(part 1 of 2)
# Autodesk Inventor assembly: CNC-FullAssembly
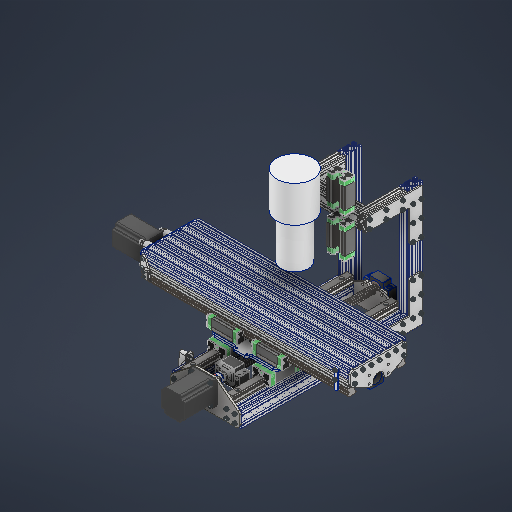
[picture p0: Inventor's stored thumbnail of the model, 512x512]
Saved by Autodesk Inventor 2026.2 (Build 302298000, 298)
## iProperties
Created: 2026-06-14
Part Number: CNC-FullAssembly
Document SubType Name: Assembly
Designer: Kenji
Mass: 17887.4 g
Surface Area: 25590.9 cm^2
Volume: 4676.24 cm^3
Density: 3.82518 g/cm^3
Author: Kenji
## Documents named in this file (45)
- C:\Users\Kenji\Documents\GitHub\DiyCNC-\CNC-FullAssembly.iam
- C:\Users\Kenji\Documents\GitHub\DiyCNC-\COTS-Parts\40x40x500mm-Extrusion.ipt
- C:\Users\Kenji\Documents\GitHub\DiyCNC-\COTS-Parts\SFU1605-BallScrewNut.iam
- C:\Users\Kenji\Documents\GitHub\DiyCNC-\COTS-Parts\DSG16H-BallScrewFixtureBlock.ipt
- C:\Users\Kenji\Documents\GitHub\DiyCNC-\COTS-Parts\SFU1605-BallScrew500mm.ipt
- C:\Users\Kenji\Documents\GitHub\DiyCNC-\COTS-Parts\BK12-BallScrewStabilizer.iam
- C:\Users\Kenji\Documents\GitHub\DiyCNC-\COTS-Parts\HGR20R-LinearRail500mm.ipt
- C:\Users\Kenji\Documents\GitHub\DiyCNC-\COTS-Parts\HGH20-LinearRailCarriage.iam
- C:\Users\Kenji\Documents\GitHub\DiyCNC-\COTS-Parts\91274A131_M5x20mm.ipt
- C:\Users\Kenji\Documents\GitHub\DiyCNC-\COTS-Parts\91290A231-M5x15mm.ipt
- C:\Users\Kenji\Documents\GitHub\DiyCNC-\COTS-Parts\Nema23-StepperMotor.ipt
- C:\Users\Kenji\Documents\GitHub\DiyCNC-\COTS-Parts\MH2025-6.35x10mmCoupler.iam
- C:\Users\Kenji\Documents\GitHub\DiyCNC-\COTS-Parts\BF12-BallScrewStabilizer2.ipt
- C:\Users\Kenji\Documents\GitHub\DiyCNC-\CNC-000-StructureGusset1.ipt
- C:\Users\Kenji\Documents\GitHub\DiyCNC-\COTS-Parts\20x40x500mm-Extrusion.ipt
- C:\Users\Kenji\Documents\GitHub\DiyCNC-\CNC-001-StructureGusset2.ipt
- C:\Users\Kenji\Documents\GitHub\DiyCNC-\CNC-002-ShimStructureGusset2.ipt
- C:\Users\Kenji\Documents\GitHub\DiyCNC-\COTS-Parts\90576A104-M5-NylockNut.ipt
- C:\Users\Kenji\Documents\GitHub\DiyCNC-\COTS-Parts\91292A195-M5x45mm.ipt
- C:\Users\Kenji\Documents\GitHub\DiyCNC-\CNC-003-StructureGusset3.ipt
- C:\Users\Kenji\Documents\GitHub\DiyCNC-\CNC-004-Nema23Shim.ipt
- C:\Users\Kenji\Documents\GitHub\DiyCNC-\COTS-Parts\91274A125-M5x8mm.ipt
- C:\Users\Kenji\Documents\GitHub\DiyCNC-\CNC-005-XAxisMount1.ipt
- C:\Users\Kenji\Documents\GitHub\DiyCNC-\COTS-Parts\91263A832-M5x10mm-Countersink.ipt
- C:\Users\Kenji\Documents\GitHub\DiyCNC-\CNC-006-XAxisMount2.ipt
- C:\Users\Kenji\Documents\GitHub\DiyCNC-\COTS-Parts\92095A495-M8-18mm-ButtonHead.ipt
- C:\Users\Kenji\Documents\GitHub\DiyCNC-\COTS-Parts\94645A210-M8-NylockNut.ipt
- C:\Users\Kenji\Documents\GitHub\DiyCNC-\COTS-Parts\20x40x500mm-Extrusion2.ipt
- C:\Users\Kenji\Documents\GitHub\DiyCNC-\COTS-Parts\20x20x500mm_Extrusion.ipt
- C:\Users\Kenji\Documents\GitHub\DiyCNC-\CNC-007-XAxisBallScrewMount.ipt
- C:\Users\Kenji\Documents\GitHub\DiyCNC-\CNC-008-XAxisNema23Mount.ipt
- C:\Users\Kenji\Documents\GitHub\DiyCNC-\CNC-009-XAxisNema23Spacer.ipt
- C:\Users\Kenji\Documents\GitHub\DiyCNC-\COTS-Parts\91290A198-M5-50mm.ipt
- C:\Users\Kenji\Documents\GitHub\DiyCNC-\COTS-Parts\3103-0001-0002-GobildaLimitSwitch.ipt
- C:\Users\Kenji\Documents\GitHub\DiyCNC-\CNC-010-XAxisLimitSwitchMount.ipt
- C:\Users\Kenji\Documents\GitHub\DiyCNC-\COTS-Parts\97763A820-M5x10mm-ButtonHead.ipt
- C:\Users\Kenji\Documents\GitHub\DiyCNC-\CNC-011-XAxisHardStop.ipt
- C:\Users\Kenji\Documents\GitHub\DiyCNC-\COTS-Parts\HGR20R-LinearRail300mm.ipt
- C:\Users\Kenji\Documents\GitHub\DiyCNC-\COTS-Parts\SFU1605-BallScrew400mm.ipt
- C:\Users\Kenji\Documents\GitHub\DiyCNC-\COTS-Parts\RouterSpindle-65mm.ipt
- C:\Users\Kenji\Documents\GitHub\DiyCNC-\COTS-Parts\90128A046-#2-.375in.ipt
- C:\Users\Kenji\Documents\GitHub\DiyCNC-\COTS-Parts\90480A003-#2-HexNut.ipt
- C:\Users\Kenji\Documents\GitHub\DiyCNC-\CNC-012-YAxisLimitSwitchMount.ipt
- C:\Users\Kenji\Documents\GitHub\DiyCNC-\COTS-Parts\20x40x100mm-Extrusion.ipt
- C:\Users\Kenji\Documents\GitHub\DiyCNC-\COTS-Parts\20x40x128mm-Extrusion.ipt
## Components (278 placed, 44 different names)
1. 40x40x500mm-Extrusion:1 — Mate:1, Mate:2, Flush:1, Flush:2, Flush:3, Angle:1, Angle:3, Angle:4, Flush:20, Flush:21, Mate:48, Mate:49, Flush:35, Mate:264, Mate:286, Flush:146, Mate:293, Tangent:7
2. 40x40x500mm-Extrusion:2 — Flush:2, Flush:3, Angle:2, Mate:39, Mate:40, Mate:41, Flush:22, Flush:23, Flush:38, Mate:290, Flush:147, Mate:294, Mate:299, Angle:12, Mate:315, Angle:13, Flush:153
3. SFU1605-BallScrewNut:1 [sub-assembly] — Mate:3, Mate:4, Mate:5, Mate:21, Mate:22, Mate:23, Mate:24, Mate:25, Mate:26, Mate:27
4. DSG16H-BallScrewFixtureBlock:1 — Mate:3, Mate:4, Mate:5, Angle:1, Flush:14, Mate:20, Angle:6, Mate:98, Mate:99
5. BK12-BallScrewStabilizer:1 [sub-assembly] — Angle:2, Mate:295, Mate:296
6. HGH20-LinearRailCarriage:1 [sub-assembly] — Flush:10, Flush:11, Mate:18, Flush:14, Mate:100, Mate:284, Mate:303, Mate:304
7. HGH20-LinearRailCarriage:2 [sub-assembly] — Flush:12, Flush:13, Mate:283, Mate:329
8. HGH20-LinearRailCarriage:3 [sub-assembly] — Flush:10, Flush:12, Mate:20, Mate:281, Mate:282, Flush:150
9. HGH20-LinearRailCarriage:4 [sub-assembly] — Flush:11, Mate:18, Flush:13, Mate:285
10. 91274A131_M5x20mm:1 — Mate:21, Mate:22, Flush:17, Flush:18
11. 91274A131_M5x20mm:2 — Mate:26, Flush:15, Flush:16
12. 91274A131_M5x20mm:3 — Mate:27, Flush:15
13. 91274A131_M5x20mm:4 — Mate:25, Flush:16, Flush:17
14. 91274A131_M5x20mm:5 — Mate:23, Flush:18, Flush:19
15. 91274A131_M5x20mm:6 — Mate:24, Flush:19
16. Nema23-StepperMotor:1 — Mate:32, Angle:3, Mate:33, Mate:59, Mate:60, Mate:61, Mate:62, Mate:63, Mate:301
17. MH2025-6.35x10mmCoupler:1 [sub-assembly] — Mate:32, Mate:33, Mate:297
18. BF12-BallScrewStabilizer2:1 — Angle:4, Mate:56, Mate:57, Mate:58, Mate:269, Mate:298
19. CNC-000-StructureGusset1:1 — Mate:39, Mate:40, Mate:41, Mate:42, Mate:43, Mate:44, Mate:45, Mate:65, Mate:77, Mate:79, Mate:265, Mate:287, Mate:291, Mate:302
20. 20x40x500mm-Extrusion:1 — Flush:20, Flush:21, Mate:71, Mate:72, Mate:73, Mate:74, Mate:75, Flush:36, Mate:293, Tangent:8, Flush:156, Flush:157, Mate:331, Flush:159, Mate:337, Mate:338, Mate:339
21. 20x40x500mm-Extrusion:2 — Flush:22, Flush:23, Mate:69, Mate:70, Mate:76, Flush:37, Mate:294, Mate:329, Mate:330, Flush:154, Flush:155, Mate:340, Mate:341
22. CNC-001-StructureGusset2:1 — Mate:48, Mate:49, Mate:51, Mate:52, Mate:53, Mate:54, Mate:55, Mate:269, Mate:299, Mate:300
23. 91290A231-M5x15mm:27 — Mate:51, Mate:52, Flush:25, Flush:26
24. 91290A231-M5x15mm:28 — Mate:54, Flush:24, Flush:25
25. 91290A231-M5x15mm:29 — Mate:55, Flush:24
26. 91290A231-M5x15mm:30 — Mate:53, Flush:26
27. CNC-002-ShimStructureGusset2:1 — Mate:56, Mate:57, Mate:58, Mate:300
28. 91274A131_M5x20mm:7 — Mate:60, Flush:29, Mate:67
29. 91274A131_M5x20mm:8 — Mate:62, Mate:63, Flush:27, Mate:68
30. 91274A131_M5x20mm:9 — Mate:59, Flush:28, Flush:29, Mate:64
31. 91274A131_M5x20mm:10 — Mate:61, Flush:27, Flush:28, Mate:66
32. 90576A104-M5-NylockNut:1 — Mate:64, Mate:65, Flush:32
33. 90576A104-M5-NylockNut:2 — Mate:66, Flush:30, Mate:78, Mate:265
34. 90576A104-M5-NylockNut:3 — Mate:68, Flush:30, Flush:31
35. 90576A104-M5-NylockNut:4 — Mate:67, Flush:31, Flush:32
36. 91292A195-M5x45mm:1 — Mate:69, Flush:33, Flush:34
37. 91292A195-M5x45mm:2 — Mate:70, Flush:34
38. 91292A195-M5x45mm:3 — Mate:72, Mate:73
39. 91292A195-M5x45mm:4 — Mate:71, Mate:74, Flush:33
40. CNC-003-StructureGusset3:1 — Mate:75, Flush:35, Flush:36, Mate:80, Mate:81, Mate:82, Mate:83
41. CNC-003-StructureGusset3:2 — Mate:76, Flush:37, Flush:38, Mate:84, Mate:85, Mate:86, Mate:87
42. CNC-004-Nema23Shim:1 — Mate:77, Mate:78, Mate:79, Mate:301
43. HGH20-LinearRailCarriage:5 [sub-assembly] — Mate:91, Mate:92, Mate:131, Mate:132, Mate:133, Flush:142
44. HGH20-LinearRailCarriage:6 [sub-assembly] — Mate:128, Mate:129, Mate:130
45. HGH20-LinearRailCarriage:7 [sub-assembly] — Mate:125, Mate:126, Mate:127
46. HGH20-LinearRailCarriage:8 [sub-assembly] — Mate:134, Mate:135, Mate:136, Mate:137, Mate:138
47. HGR20R-LinearRail500mm:3 — Flush:50, Mate:137, Mate:138, Mate:202, Mate:226, Mate:314
48. HGR20R-LinearRail500mm:4 — Mate:91, Mate:92, Flush:50, Flush:106, Flush:107, Mate:199, Flush:119, Angle:10, Mate:224, Mate:225, Flush:142, Mate:313
49. DSG16H-BallScrewFixtureBlock:2 — Angle:6, Mate:94, Mate:95, Mate:96, Mate:97, Mate:121, Mate:122, Mate:123
50. SFU1605-BallScrewNut:2 [sub-assembly] — Mate:94, Mate:95, Mate:96, Mate:139, Mate:140, Mate:141, Mate:142, Mate:143, Mate:144, Mate:145
51. SFU1605-BallScrew500mm:2 — Mate:97, Mate:203, Mate:204, Mate:205, Mate:207, Mate:209, Mate:256
52. CNC-005-XAxisMount1:1 — Mate:98, Mate:99, Mate:100, Mate:101, Flush:53, Mate:102, Mate:103, Mate:104, Mate:105, Mate:106, Mate:107, Mate:108, Flush:57, Flush:58, Flush:59, Flush:60, Mate:109, Mate:110, Mate:111, Mate:112, Flush:61, Flush:63, Mate:113, Mate:114, Mate:115, Mate:116, Flush:65, Flush:66, Flush:67, Flush:68, Mate:117, Mate:118, Mate:119, Mate:120, Flush:69, Flush:70, Flush:71, Flush:72, Mate:124, Angle:7, Mate:166, Mate:177, Mate:179, Mate:181, Mate:183, Mate:186, Mate:187, Mate:190, Mate:191, Mate:282, Mate:283, Mate:285
53. 91263A832-M5x10mm-Countersink:1 — Mate:101, Flush:53, Flush:56
54. 91263A832-M5x10mm-Countersink:2 — Mate:104, Flush:55, Mate:281
55. 91263A832-M5x10mm-Countersink:3 — Mate:102, Flush:54, Flush:55, Flush:56
56. 91263A832-M5x10mm-Countersink:4 — Mate:103, Flush:54
57. 91263A832-M5x10mm-Countersink:5 — Mate:105, Flush:59
58. 91263A832-M5x10mm-Countersink:6 — Mate:106, Flush:58, Mate:284
59. 91263A832-M5x10mm-Countersink:7 — Mate:108, Flush:57
60. 91263A832-M5x10mm-Countersink:8 — Mate:107, Flush:60
61. 91263A832-M5x10mm-Countersink:9 — Mate:112, Flush:62
62. 91263A832-M5x10mm-Countersink:10 — Mate:111, Flush:61, Flush:62
63. 91263A832-M5x10mm-Countersink:11 — Mate:109, Flush:63, Flush:64
64. 91263A832-M5x10mm-Countersink:12 — Mate:110, Flush:64
65. 91263A832-M5x10mm-Countersink:13 — Mate:113, Flush:65
66. 91263A832-M5x10mm-Countersink:14 — Mate:116, Flush:67
67. 91263A832-M5x10mm-Countersink:15 — Mate:115, Flush:66
68. 91263A832-M5x10mm-Countersink:16 — Mate:114, Flush:68
69. 91263A832-M5x10mm-Countersink:17 — Mate:118, Flush:71
70. 91263A832-M5x10mm-Countersink:18 — Mate:119, Flush:69
71. 91263A832-M5x10mm-Countersink:19 — Mate:117, Flush:72
72. 91263A832-M5x10mm-Countersink:20 — Mate:120, Flush:70
73. CNC-006-XAxisMount2:1 — Mate:121, Mate:122, Mate:123, Mate:124, Angle:7, Mate:125, Mate:126, Mate:127, Mate:128, Mate:129, Mate:130, Mate:131, Mate:132, Mate:133, Mate:134, Mate:135, Mate:136, Mate:146, Mate:147, Mate:148, Mate:149, Flush:78, Flush:79, Flush:81, Mate:150, Mate:151, Mate:152, Mate:153, Flush:82, Flush:83, Flush:84, Flush:85, Mate:154, Mate:155, Mate:156, Mate:157, Flush:86, Flush:87, Mate:158, Mate:159, Mate:160, Mate:161, Flush:90, Flush:91, Flush:92, Flush:93, Mate:162, Mate:163, Mate:164, Mate:165, Flush:94, Flush:95, Flush:96, Flush:97, Mate:166, Mate:167, Mate:168, Mate:169, Mate:170, Mate:171, Mate:172, Mate:173, Mate:174, Mate:175
74. 91274A131_M5x20mm:11 — Mate:139, Mate:140, Flush:74, Flush:75
75. 91274A131_M5x20mm:12 — Mate:145, Flush:76, Flush:77
76. 91274A131_M5x20mm:13 — Mate:144, Flush:77
77. 91274A131_M5x20mm:14 — Mate:141, Flush:73, Flush:74
78. 91274A131_M5x20mm:15 — Mate:143, Flush:75
79. 91274A131_M5x20mm:16 — Mate:142, Flush:73, Flush:76
80. 91263A832-M5x10mm-Countersink:21 — Mate:149, Flush:78
81. 91263A832-M5x10mm-Countersink:22 — Mate:146, Flush:80
82. 91263A832-M5x10mm-Countersink:23 — Mate:147, Flush:79, Flush:80
83. 91263A832-M5x10mm-Countersink:24 — Mate:148, Flush:81
84. 91263A832-M5x10mm-Countersink:25 — Mate:150, Flush:85
85. 91263A832-M5x10mm-Countersink:26 — Mate:153, Flush:83
86. 91263A832-M5x10mm-Countersink:27 — Mate:151, Flush:82
87. 91263A832-M5x10mm-Countersink:28 — Mate:152, Flush:84
88. 91263A832-M5x10mm-Countersink:29 — Mate:156, Flush:87, Flush:88
89. 91263A832-M5x10mm-Countersink:30 — Mate:155, Flush:89
90. 91263A832-M5x10mm-Countersink:31 — Mate:154, Flush:88, Flush:89
91. 91263A832-M5x10mm-Countersink:32 — Mate:157, Flush:86
92. 91263A832-M5x10mm-Countersink:33 — Mate:159, Flush:93
93. 91263A832-M5x10mm-Countersink:34 — Mate:160, Flush:91
94. 91263A832-M5x10mm-Countersink:35 — Mate:158, Flush:92
95. 91263A832-M5x10mm-Countersink:36 — Mate:161, Flush:90
96. 91263A832-M5x10mm-Countersink:37 — Mate:164, Flush:95
97. 91263A832-M5x10mm-Countersink:38 — Mate:162, Flush:96
98. 91263A832-M5x10mm-Countersink:39 — Mate:163, Flush:97
99. 91263A832-M5x10mm-Countersink:40 — Mate:165, Flush:94
100. 92095A495-M8-18mm-ButtonHead:1 — Mate:167, Flush:98, Flush:99, Flush:102, Mate:176
101. 92095A495-M8-18mm-ButtonHead:2 — Mate:168, Flush:99, Flush:104, Mate:178
102. 92095A495-M8-18mm-ButtonHead:3 — Mate:169, Mate:170, Flush:98, Flush:100, Mate:180
103. 92095A495-M8-18mm-ButtonHead:8 — Mate:171, Flush:100, Mate:182
104. 92095A495-M8-18mm-ButtonHead:9 — Mate:174, Flush:103, Flush:104, Mate:188
105. 92095A495-M8-18mm-ButtonHead:10 — Mate:175, Flush:103, Mate:189
106. 92095A495-M8-18mm-ButtonHead:11 — Mate:172, Flush:101, Flush:102, Mate:184
107. 92095A495-M8-18mm-ButtonHead:12 — Mate:173, Flush:101, Mate:185
108. 94645A210-M8-NylockNut:1 — Mate:176, Mate:177
109. 94645A210-M8-NylockNut:2 — Mate:178, Mate:179
110. 94645A210-M8-NylockNut:3 — Mate:180, Mate:181
111. 94645A210-M8-NylockNut:4 — Mate:182, Mate:183
112. 94645A210-M8-NylockNut:5 — Mate:184, Mate:187
113. 94645A210-M8-NylockNut:6 — Mate:185, Mate:186
114. 94645A210-M8-NylockNut:7 — Mate:188, Mate:191
115. 94645A210-M8-NylockNut:8 — Mate:189, Mate:190
116. 20x40x500mm-Extrusion2:1 — Flush:106, Flush:107, Flush:108, Mate:193, Flush:109, Flush:116, Flush:117, Mate:200, Mate:211, Mate:212, Mate:213, Angle:11, Tangent:2, Flush:143, Tangent:4, Mate:270
117. 20x40x500mm-Extrusion2:2 — Flush:108, Mate:193, Flush:109, Flush:110, Flush:111, Mate:194, Angle:8, Angle:9
118. 20x40x500mm-Extrusion2:3 — Flush:110, Flush:111, Mate:194, Mate:201, Flush:118, Mate:228, Mate:229
119. 20x20x500mm_Extrusion:3 — Flush:116, Mate:199, Flush:117, Mate:200, Tangent:3, Tangent:5, Flush:144, Mate:312
120. 20x40x500mm-Extrusion2:4 — Mate:201, Flush:118, Mate:202, Mate:227, Mate:276
121. BF12-BallScrewStabilizer2:2 — Mate:203, Mate:204, Flush:119, Angle:8
122. Nema23-StepperMotor:2 — Mate:205, Angle:9, Mate:206, Mate:208, Mate:243, Mate:244, Mate:245, Mate:246, Mate:247
123. MH2025-6.35x10mmCoupler:2 [sub-assembly] — Mate:206, Mate:207, Mate:208, Mate:240
124. BK12-BallScrewStabilizer:2 [sub-assembly] — Mate:209, Angle:10, Mate:256
125. CNC-007-XAxisBallScrewMount:1 — Mate:211, Mate:212, Mate:213, Mate:214, Mate:215, Mate:216, Mate:217, Mate:218, Mate:219, Mate:220, Mate:221, Mate:222, Mate:223
126. 91290A231-M5x15mm:31 — Mate:219, Flush:123, Flush:124
127. 91290A231-M5x15mm:32 — Mate:218, Flush:122, Flush:123, Flush:125, Flush:127
128. 91290A231-M5x15mm:33 — Mate:215, Flush:120, Flush:121
129. 91290A231-M5x15mm:34 — Mate:216, Flush:120
130. 91290A231-M5x15mm:35 — Mate:220, Flush:124
131. 91290A231-M5x15mm:36 — Mate:214, Mate:221, Flush:125, Flush:126
132. 91290A231-M5x15mm:37 — Mate:217, Flush:121, Flush:122
133. 91290A231-M5x15mm:38 — Mate:222, Flush:126
134. 91290A231-M5x15mm:39 — Mate:223, Flush:127
135. CNC-008-XAxisNema23Mount:1 — Mate:227, Mate:228, Mate:229, Mate:230, Mate:231, Mate:232, Mate:233, Mate:234, Mate:235, Mate:236, Mate:237, Mate:238, Mate:239, Mate:241, Mate:242, Mate:252, Mate:253, Mate:254, Mate:255
136. 91290A231-M5x15mm:58 — Mate:233, Flush:133, Flush:134
137. 91290A231-M5x15mm:59 — Mate:231, Flush:134, Flush:135
138. 91290A231-M5x15mm:60 — Mate:232, Flush:136
139. 91290A231-M5x15mm:61 — Mate:234, Flush:132, Flush:133
140. 91290A231-M5x15mm:62 — Mate:235, Flush:131, Flush:132
141. 91290A231-M5x15mm:63 — Mate:238, Mate:239, Flush:129
142. 91290A231-M5x15mm:64 — Mate:230, Flush:135, Flush:136
143. 91290A231-M5x15mm:65 — Mate:237, Flush:129, Flush:130
144. 91290A231-M5x15mm:66 — Mate:236, Flush:130, Flush:131
145. CNC-009-XAxisNema23Spacer:1 — Mate:240, Mate:241, Mate:242
146. 91290A198-M5-50mm:1 — Mate:244, Flush:138, Mate:248
147. 91290A198-M5-50mm:2 — Mate:243, Flush:138, Flush:139, Mate:250
148. 91290A198-M5-50mm:3 — Mate:245, Flush:137, Flush:139, Mate:251
149. 91290A198-M5-50mm:4 — Mate:246, Mate:247, Flush:137, Mate:249
150. 90576A104-M5-NylockNut:5 — Mate:251, Mate:252
151. 90576A104-M5-NylockNut:6 — Mate:248, Mate:254
152. 90576A104-M5-NylockNut:7 — Mate:250, Mate:255
153. 90576A104-M5-NylockNut:8 — Mate:249, Mate:253
154. 3103-0001-0002-GobildaLimitSwitch:1 — Angle:11, Mate:258, Mate:259, Mate:305, Mate:306, Mate:310
155. CNC-010-XAxisLimitSwitchMount:1 — Tangent:2, Mate:258, Mate:259, Mate:260, Mate:261, Mate:262, Mate:263, Tangent:3, Flush:143, Mate:307, Mate:308, Mate:312
156. 97763A820-M5x10mm-ButtonHead:1 — Mate:262, Mate:263
157. 97763A820-M5x10mm-ButtonHead:2 — Mate:260, Mate:261
158. CNC-011-XAxisHardStop:1 — Tangent:4, Tangent:5, Mate:270, Flush:144, Mate:271, Mate:272, Mate:273, Mate:274
159. 91274A125-M5x8mm:25 — Mate:271, Mate:272, Flush:145
160. 91274A125-M5x8mm:26 — Mate:273, Flush:145, Mate:275
161. CNC-011-XAxisHardStop:2 — Mate:274, Mate:275, Mate:276, Mate:277, Mate:278, Mate:279, Mate:280
162. 91274A125-M5x8mm:27 — Mate:277, Mate:280
163. 91274A125-M5x8mm:28 — Mate:278, Mate:279
164. HGR20R-LinearRail300mm:1 — Mate:290, Mate:291, Flush:147, Mate:292
165. HGR20R-LinearRail300mm:2 — Mate:286, Flush:146, Mate:287, Mate:288, Mate:289, Mate:303, Mate:304
166. SFU1605-BallScrew400mm:1 — Mate:295, Mate:296, Mate:297, Mate:298
167. RouterSpindle-65mm:1 — Tangent:7, Tangent:8
168. 90128A046-#2-.375in:1 — Mate:305, Mate:308, Mate:311
169. 90128A046-#2-.375in:2 — Mate:306, Mate:307, Mate:309
170. 90480A003-#2-HexNut:1 — Mate:309, Mate:310, Flush:149
171. 90480A003-#2-HexNut:2 — Mate:311, Flush:149
172. 3103-0001-0002-GobildaLimitSwitch:2 — Angle:12, Flush:150, Mate:315, Mate:316, Mate:318, Mate:321, Mate:323, Mate:324, Mate:325
173. CNC-012-YAxisLimitSwitchMount:1 — Mate:316, Mate:318, Angle:13, Mate:319, Angle:14, Mate:320, Angle:15, Mate:322, Mate:326, Mate:327, Mate:328, Flush:153
174. 90480A003-#2-HexNut:3 — Mate:319, Angle:14, Mate:320
175. 90480A003-#2-HexNut:4 — Mate:321, Angle:15, Mate:322
176. 90128A046-#2-.375in:3 — Mate:323, Flush:151
177. 90128A046-#2-.375in:4 — Mate:324, Mate:325, Flush:151
178. 97763A820-M5x10mm-ButtonHead:3 — Mate:326, Flush:152
179. 97763A820-M5x10mm-ButtonHead:4 — Mate:327, Mate:328, Flush:152
180. 20x40x100mm-Extrusion:3 — Mate:330, Flush:154, Flush:155, Mate:335, Mate:336, Flush:160, Flush:161
181. 20x40x100mm-Extrusion:4 — Flush:156, Flush:157, Mate:331, Mate:332, Flush:158
182. CNC-003-StructureGusset3:3 — Mate:332, Flush:158, Flush:159, Mate:333, Mate:334, Mate:342, Mate:343, Mate:344
183. CNC-003-StructureGusset3:4 — Mate:333, Mate:334, Mate:335, Mate:345, Mate:346, Mate:347, Mate:348
184. 20x40x128mm-Extrusion:1 — Mate:336, Flush:160, Flush:161, Mate:349, Angle:16, Flush:168, Mate:350
185. 91292A195-M5x45mm:5 — Mate:337, Mate:338, Flush:164
186. 91292A195-M5x45mm:6 — Mate:341, Flush:162
187. 91292A195-M5x45mm:7 — Mate:339, Flush:163, Flush:164
188. 91292A195-M5x45mm:8 — Mate:340, Flush:162, Flush:163
189. HGH20-LinearRailCarriage:9 [sub-assembly] — Mate:349, Angle:16, Flush:166, Flush:167, Mate:351
190. HGH20-LinearRailCarriage:10 [sub-assembly] — Flush:166, Flush:167, Flush:168, Mate:350, Mate:351
191. 91290A231-M5x15mm:20 — Mate:44, Mate:45
192. 91290A231-M5x15mm:21
193. 91290A231-M5x15mm:22 — Mate:264
194. 91290A231-M5x15mm:23 — Mate:302
195. 91290A231-M5x15mm:19 — Mate:42, Mate:43
196. 91290A231-M5x15mm:24
197. 91290A231-M5x15mm:25
198. 91290A231-M5x15mm:26
199. 91274A125-M5x8mm:1 — Mate:80, Mate:81
200. 91274A125-M5x8mm:2
201. 91274A125-M5x8mm:3
202. 91274A125-M5x8mm:4
203. 91274A125-M5x8mm:5
204. 91274A125-M5x8mm:6
205. 91274A125-M5x8mm:7 — Mate:82, Mate:83
206. 91274A125-M5x8mm:8
207. 91274A125-M5x8mm:9
208. 91274A125-M5x8mm:10
209. 91274A125-M5x8mm:11
210. 91274A125-M5x8mm:12
211. 91274A125-M5x8mm:13 — Mate:84, Mate:85
212. 91274A125-M5x8mm:14
213. 91274A125-M5x8mm:15
214. 91274A125-M5x8mm:16
215. 91274A125-M5x8mm:17
216. 91274A125-M5x8mm:18
217. 91274A125-M5x8mm:19 — Mate:86, Mate:87
218. 91274A125-M5x8mm:20
219. 91274A125-M5x8mm:21
220. 91274A125-M5x8mm:22
221. 91274A125-M5x8mm:23
222. 91274A125-M5x8mm:24
223. 91290A231-M5x15mm:41 — Mate:226, Flush:128
224. 91290A231-M5x15mm:40 — Mate:224, Mate:225, Flush:128
225. 91290A231-M5x15mm:67
226. 91290A231-M5x15mm:68
227. 91290A231-M5x15mm:69
228. 91290A231-M5x15mm:70
229. 91290A231-M5x15mm:71
230. 91290A231-M5x15mm:72
231. 91290A231-M5x15mm:73
232. 91290A231-M5x15mm:74
233. 91290A231-M5x15mm:75
234. 91290A231-M5x15mm:76
235. 91290A231-M5x15mm:77
236. 91290A231-M5x15mm:78
237. 91290A231-M5x15mm:79
238. 91290A231-M5x15mm:80
239. 91290A231-M5x15mm:81 — Mate:314
240. 91290A231-M5x15mm:82 — Mate:313
241. 91290A231-M5x15mm:83 — Mate:292, Flush:148
242. 91290A231-M5x15mm:1 — Mate:288, Mate:289, Flush:148
243. 91290A231-M5x15mm:84
244. 91290A231-M5x15mm:85
245. 91290A231-M5x15mm:86
246. 91290A231-M5x15mm:87
247. 91290A231-M5x15mm:88
248. 91290A231-M5x15mm:89
249. 91290A231-M5x15mm:90
250. 91290A231-M5x15mm:91
251. 91290A231-M5x15mm:92
252. 91290A231-M5x15mm:93
253. 91290A231-M5x15mm:94
254. 91290A231-M5x15mm:95
255. 91274A125-M5x8mm:29 — Mate:342, Mate:343, Flush:165
256. 91274A125-M5x8mm:33
257. 91274A125-M5x8mm:34
258. 91274A125-M5x8mm:35
259. 91274A125-M5x8mm:36
260. 91274A125-M5x8mm:37
261. 91274A125-M5x8mm:30 — Mate:344, Flush:165
262. 91274A125-M5x8mm:38
263. 91274A125-M5x8mm:39
264. 91274A125-M5x8mm:40
265. 91274A125-M5x8mm:41
266. 91274A125-M5x8mm:42
267. 91274A125-M5x8mm:31 — Mate:345, Mate:346
268. 91274A125-M5x8mm:43
269. 91274A125-M5x8mm:44
270. 91274A125-M5x8mm:45
271. 91274A125-M5x8mm:46
272. 91274A125-M5x8mm:47
273. 91274A125-M5x8mm:32 — Mate:347, Mate:348
274. 91274A125-M5x8mm:48
275. 91274A125-M5x8mm:49
276. 91274A125-M5x8mm:50
277. 91274A125-M5x8mm:51
278. 91274A125-M5x8mm:52
## Component patterns: (4 elements, first: 91290A231-M5x15mm:20), (4 elements, first: 91290A231-M5x15mm:19), (6 elements, first: 91274A125-M5x8mm:1), (6 elements, first: 91274A125-M5x8mm:7), (6 elements, first: 91274A125-M5x8mm:13), (6 elements, first: 91274A125-M5x8mm:19), (9 elements, first: 91290A231-M5x15mm:41 + 91290A231-M5x15mm:40), (7 elements, first: 91290A231-M5x15mm:83 + 91290A231-M5x15mm:1), (6 elements, first: 91274A125-M5x8mm:29), (6 elements, first: 91274A125-M5x8mm:30), (6 elements, first: 91274A125-M5x8mm:31), (6 elements, first: 91274A125-M5x8mm:32)
## Relationships (474: Mate 311, Flush 142, Angle 15, Tangent 6)
- Mate:1 (-20 mm): 40x40x500mm-Extrusion:1
- Mate:2 (-20 mm): 40x40x500mm-Extrusion:1
- Flush:1 (-250 mm): 40x40x500mm-Extrusion:1
- Flush:2: 40x40x500mm-Extrusion:1 ↔ 40x40x500mm-Extrusion:2
- Flush:3: 40x40x500mm-Extrusion:1 ↔ 40x40x500mm-Extrusion:2
- Mate:3: SFU1605-BallScrewNut:1 ↔ DSG16H-BallScrewFixtureBlock:1
- Mate:4: SFU1605-BallScrewNut:1 ↔ DSG16H-BallScrewFixtureBlock:1
- Mate:5: SFU1605-BallScrewNut:1 ↔ DSG16H-BallScrewFixtureBlock:1
- Angle:1 (0 deg): 40x40x500mm-Extrusion:1 ↔ DSG16H-BallScrewFixtureBlock:1
- Angle:2 (0 deg): 40x40x500mm-Extrusion:2 ↔ BK12-BallScrewStabilizer:1
- Flush:10: HGH20-LinearRailCarriage:1 ↔ HGH20-LinearRailCarriage:3
- Flush:11: HGH20-LinearRailCarriage:1 ↔ HGH20-LinearRailCarriage:4
- Mate:18 (40 mm): HGH20-LinearRailCarriage:1 ↔ HGH20-LinearRailCarriage:4
- Flush:12: HGH20-LinearRailCarriage:2 ↔ HGH20-LinearRailCarriage:3
- Flush:13: HGH20-LinearRailCarriage:2 ↔ HGH20-LinearRailCarriage:4
- Flush:14: DSG16H-BallScrewFixtureBlock:1 ↔ HGH20-LinearRailCarriage:1
- Mate:20: DSG16H-BallScrewFixtureBlock:1 ↔ HGH20-LinearRailCarriage:3
- Mate:21: SFU1605-BallScrewNut:1 ↔ 91274A131_M5x20mm:1
- Mate:22: SFU1605-BallScrewNut:1 ↔ 91274A131_M5x20mm:1
- Mate:23: SFU1605-BallScrewNut:1 ↔ 91274A131_M5x20mm:5
- Mate:24: SFU1605-BallScrewNut:1 ↔ 91274A131_M5x20mm:6
- Mate:25: SFU1605-BallScrewNut:1 ↔ 91274A131_M5x20mm:4
- Mate:26: SFU1605-BallScrewNut:1 ↔ 91274A131_M5x20mm:2
- Mate:27: SFU1605-BallScrewNut:1 ↔ 91274A131_M5x20mm:3
- Flush:15: 91274A131_M5x20mm:2 ↔ 91274A131_M5x20mm:3
- Flush:16: 91274A131_M5x20mm:2 ↔ 91274A131_M5x20mm:4
- Flush:17: 91274A131_M5x20mm:1 ↔ 91274A131_M5x20mm:4
- Flush:18: 91274A131_M5x20mm:1 ↔ 91274A131_M5x20mm:5
- Flush:19: 91274A131_M5x20mm:5 ↔ 91274A131_M5x20mm:6
- Mate:32: Nema23-StepperMotor:1 ↔ MH2025-6.35x10mmCoupler:1
- Angle:3 (0 deg): 40x40x500mm-Extrusion:1 ↔ Nema23-StepperMotor:1
- Mate:33 (2 mm): Nema23-StepperMotor:1 ↔ MH2025-6.35x10mmCoupler:1
- Angle:4 (0 deg): 40x40x500mm-Extrusion:1 ↔ BF12-BallScrewStabilizer2:1
- Mate:39: 40x40x500mm-Extrusion:2 ↔ CNC-000-StructureGusset1:1
- Mate:40: 40x40x500mm-Extrusion:2 ↔ CNC-000-StructureGusset1:1
- Mate:41: 40x40x500mm-Extrusion:2 ↔ CNC-000-StructureGusset1:1
- Mate:42: CNC-000-StructureGusset1:1 ↔ 91290A231-M5x15mm:19
- Mate:43: CNC-000-StructureGusset1:1 ↔ 91290A231-M5x15mm:19
- Mate:44: CNC-000-StructureGusset1:1 ↔ 91290A231-M5x15mm:20
- Mate:45: CNC-000-StructureGusset1:1 ↔ 91290A231-M5x15mm:20
- Flush:20: 40x40x500mm-Extrusion:1 ↔ 20x40x500mm-Extrusion:1
- Flush:21: 40x40x500mm-Extrusion:1 ↔ 20x40x500mm-Extrusion:1
- Flush:22: 40x40x500mm-Extrusion:2 ↔ 20x40x500mm-Extrusion:2
- Flush:23: 40x40x500mm-Extrusion:2 ↔ 20x40x500mm-Extrusion:2
- Mate:48: 40x40x500mm-Extrusion:1 ↔ CNC-001-StructureGusset2:1
- Mate:49: 40x40x500mm-Extrusion:1 ↔ CNC-001-StructureGusset2:1
- Mate:51: CNC-001-StructureGusset2:1 ↔ 91290A231-M5x15mm:27
- Mate:52: CNC-001-StructureGusset2:1 ↔ 91290A231-M5x15mm:27
- Mate:53: CNC-001-StructureGusset2:1 ↔ 91290A231-M5x15mm:30
- Mate:54: CNC-001-StructureGusset2:1 ↔ 91290A231-M5x15mm:28
- Mate:55: CNC-001-StructureGusset2:1 ↔ 91290A231-M5x15mm:29
- Flush:24: 91290A231-M5x15mm:28 ↔ 91290A231-M5x15mm:29
- Flush:25: 91290A231-M5x15mm:27 ↔ 91290A231-M5x15mm:28
- Flush:26: 91290A231-M5x15mm:27 ↔ 91290A231-M5x15mm:30
- Mate:56: BF12-BallScrewStabilizer2:1 ↔ CNC-002-ShimStructureGusset2:1
- Mate:57: BF12-BallScrewStabilizer2:1 ↔ CNC-002-ShimStructureGusset2:1
- Mate:58: BF12-BallScrewStabilizer2:1 ↔ CNC-002-ShimStructureGusset2:1
- Mate:59: Nema23-StepperMotor:1 ↔ 91274A131_M5x20mm:9
- Mate:60: Nema23-StepperMotor:1 ↔ 91274A131_M5x20mm:7
- Mate:61: Nema23-StepperMotor:1 ↔ 91274A131_M5x20mm:10
- Mate:62: Nema23-StepperMotor:1 ↔ 91274A131_M5x20mm:8
- Mate:63: Nema23-StepperMotor:1 ↔ 91274A131_M5x20mm:8
- Flush:27: 91274A131_M5x20mm:8 ↔ 91274A131_M5x20mm:10
- Flush:28: 91274A131_M5x20mm:9 ↔ 91274A131_M5x20mm:10
- Flush:29: 91274A131_M5x20mm:7 ↔ 91274A131_M5x20mm:9
- Mate:64: 91274A131_M5x20mm:9 ↔ 90576A104-M5-NylockNut:1
- Mate:65: CNC-000-StructureGusset1:1 ↔ 90576A104-M5-NylockNut:1
- Mate:66: 91274A131_M5x20mm:10 ↔ 90576A104-M5-NylockNut:2
- Mate:67: 91274A131_M5x20mm:7 ↔ 90576A104-M5-NylockNut:4
- Mate:68: 91274A131_M5x20mm:8 ↔ 90576A104-M5-NylockNut:3
- Flush:30: 90576A104-M5-NylockNut:2 ↔ 90576A104-M5-NylockNut:3
- Flush:31: 90576A104-M5-NylockNut:3 ↔ 90576A104-M5-NylockNut:4
- Flush:32: 90576A104-M5-NylockNut:1 ↔ 90576A104-M5-NylockNut:4
- Mate:69: 20x40x500mm-Extrusion:2 ↔ 91292A195-M5x45mm:1
- Mate:70: 20x40x500mm-Extrusion:2 ↔ 91292A195-M5x45mm:2
- Mate:71: 20x40x500mm-Extrusion:1 ↔ 91292A195-M5x45mm:4
- Mate:72: 20x40x500mm-Extrusion:1 ↔ 91292A195-M5x45mm:3
- Mate:73: 20x40x500mm-Extrusion:1 ↔ 91292A195-M5x45mm:3
- Mate:74: 20x40x500mm-Extrusion:1 ↔ 91292A195-M5x45mm:4
- Flush:33: 91292A195-M5x45mm:1 ↔ 91292A195-M5x45mm:4
- Flush:34: 91292A195-M5x45mm:1 ↔ 91292A195-M5x45mm:2
- Mate:75: 20x40x500mm-Extrusion:1 ↔ CNC-003-StructureGusset3:1
- Flush:35 (4.225 mm): 40x40x500mm-Extrusion:1 ↔ CNC-003-StructureGusset3:1
- Flush:36 (-4.225 mm): 20x40x500mm-Extrusion:1 ↔ CNC-003-StructureGusset3:1
- Mate:76: 20x40x500mm-Extrusion:2 ↔ CNC-003-StructureGusset3:2
- Flush:37 (-4.225 mm): 20x40x500mm-Extrusion:2 ↔ CNC-003-StructureGusset3:2
- Flush:38 (4.225 mm): 40x40x500mm-Extrusion:2 ↔ CNC-003-StructureGusset3:2
- Mate:77: CNC-000-StructureGusset1:1 ↔ CNC-004-Nema23Shim:1
- Mate:78: 90576A104-M5-NylockNut:2 ↔ CNC-004-Nema23Shim:1
- Mate:79: CNC-000-StructureGusset1:1 ↔ CNC-004-Nema23Shim:1
- Mate:80: CNC-003-StructureGusset3:1 ↔ 91274A125-M5x8mm:1
- Mate:81: CNC-003-StructureGusset3:1 ↔ 91274A125-M5x8mm:1
- Mate:82: CNC-003-StructureGusset3:1 ↔ 91274A125-M5x8mm:7
- Mate:83: CNC-003-StructureGusset3:1 ↔ 91274A125-M5x8mm:7
- Mate:84: CNC-003-StructureGusset3:2 ↔ 91274A125-M5x8mm:13
- Mate:85: CNC-003-StructureGusset3:2 ↔ 91274A125-M5x8mm:13
- Mate:86: CNC-003-StructureGusset3:2 ↔ 91274A125-M5x8mm:19
- Mate:87: CNC-003-StructureGusset3:2 ↔ 91274A125-M5x8mm:19
- Mate:91: HGH20-LinearRailCarriage:5 ↔ HGR20R-LinearRail500mm:4
- Mate:92: HGH20-LinearRailCarriage:5 ↔ HGR20R-LinearRail500mm:4
- Flush:50: HGR20R-LinearRail500mm:3 ↔ HGR20R-LinearRail500mm:4
- Angle:6 (180 deg): DSG16H-BallScrewFixtureBlock:1 ↔ DSG16H-BallScrewFixtureBlock:2
- Mate:94: DSG16H-BallScrewFixtureBlock:2 ↔ SFU1605-BallScrewNut:2
- Mate:95: DSG16H-BallScrewFixtureBlock:2 ↔ SFU1605-BallScrewNut:2
- Mate:96: DSG16H-BallScrewFixtureBlock:2 ↔ SFU1605-BallScrewNut:2
- Mate:97: DSG16H-BallScrewFixtureBlock:2 ↔ SFU1605-BallScrew500mm:2
- Mate:98: DSG16H-BallScrewFixtureBlock:1 ↔ CNC-005-XAxisMount1:1
- Mate:99: DSG16H-BallScrewFixtureBlock:1 ↔ CNC-005-XAxisMount1:1
- Mate:100: HGH20-LinearRailCarriage:1 ↔ CNC-005-XAxisMount1:1
- Mate:101: CNC-005-XAxisMount1:1 ↔ 91263A832-M5x10mm-Countersink:1
- Flush:53: CNC-005-XAxisMount1:1 ↔ 91263A832-M5x10mm-Countersink:1
- Mate:102: CNC-005-XAxisMount1:1 ↔ 91263A832-M5x10mm-Countersink:3
- Mate:103: CNC-005-XAxisMount1:1 ↔ 91263A832-M5x10mm-Countersink:4
- Mate:104: CNC-005-XAxisMount1:1 ↔ 91263A832-M5x10mm-Countersink:2
- Flush:54: 91263A832-M5x10mm-Countersink:3 ↔ 91263A832-M5x10mm-Countersink:4
- Flush:55: 91263A832-M5x10mm-Countersink:2 ↔ 91263A832-M5x10mm-Countersink:3
- Flush:56: 91263A832-M5x10mm-Countersink:1 ↔ 91263A832-M5x10mm-Countersink:3
- Mate:105: CNC-005-XAxisMount1:1 ↔ 91263A832-M5x10mm-Countersink:5
- Mate:106: CNC-005-XAxisMount1:1 ↔ 91263A832-M5x10mm-Countersink:6
- Mate:107: CNC-005-XAxisMount1:1 ↔ 91263A832-M5x10mm-Countersink:8
- Mate:108: CNC-005-XAxisMount1:1 ↔ 91263A832-M5x10mm-Countersink:7
- Flush:57: CNC-005-XAxisMount1:1 ↔ 91263A832-M5x10mm-Countersink:7
- Flush:58: CNC-005-XAxisMount1:1 ↔ 91263A832-M5x10mm-Countersink:6
- Flush:59: CNC-005-XAxisMount1:1 ↔ 91263A832-M5x10mm-Countersink:5
- Flush:60: CNC-005-XAxisMount1:1 ↔ 91263A832-M5x10mm-Countersink:8
- Mate:109: CNC-005-XAxisMount1:1 ↔ 91263A832-M5x10mm-Countersink:11
- Mate:110: CNC-005-XAxisMount1:1 ↔ 91263A832-M5x10mm-Countersink:12
- Mate:111: CNC-005-XAxisMount1:1 ↔ 91263A832-M5x10mm-Countersink:10
- Mate:112: CNC-005-XAxisMount1:1 ↔ 91263A832-M5x10mm-Countersink:9
- Flush:61: CNC-005-XAxisMount1:1 ↔ 91263A832-M5x10mm-Countersink:10
- Flush:62: 91263A832-M5x10mm-Countersink:9 ↔ 91263A832-M5x10mm-Countersink:10
- Flush:63: CNC-005-XAxisMount1:1 ↔ 91263A832-M5x10mm-Countersink:11
- Flush:64: 91263A832-M5x10mm-Countersink:11 ↔ 91263A832-M5x10mm-Countersink:12
- Mate:113: CNC-005-XAxisMount1:1 ↔ 91263A832-M5x10mm-Countersink:13
- Mate:114: CNC-005-XAxisMount1:1 ↔ 91263A832-M5x10mm-Countersink:16
- Mate:115: CNC-005-XAxisMount1:1 ↔ 91263A832-M5x10mm-Countersink:15
- Mate:116: CNC-005-XAxisMount1:1 ↔ 91263A832-M5x10mm-Countersink:14
- Flush:65: CNC-005-XAxisMount1:1 ↔ 91263A832-M5x10mm-Countersink:13
- Flush:66: CNC-005-XAxisMount1:1 ↔ 91263A832-M5x10mm-Countersink:15
- Flush:67: CNC-005-XAxisMount1:1 ↔ 91263A832-M5x10mm-Countersink:14
- Flush:68: CNC-005-XAxisMount1:1 ↔ 91263A832-M5x10mm-Countersink:16
- Mate:117: CNC-005-XAxisMount1:1 ↔ 91263A832-M5x10mm-Countersink:19
- Mate:118: CNC-005-XAxisMount1:1 ↔ 91263A832-M5x10mm-Countersink:17
- Mate:119: CNC-005-XAxisMount1:1 ↔ 91263A832-M5x10mm-Countersink:18
- Mate:120: CNC-005-XAxisMount1:1 ↔ 91263A832-M5x10mm-Countersink:20
- Flush:69: CNC-005-XAxisMount1:1 ↔ 91263A832-M5x10mm-Countersink:18
- Flush:70: CNC-005-XAxisMount1:1 ↔ 91263A832-M5x10mm-Countersink:20
- Flush:71: CNC-005-XAxisMount1:1 ↔ 91263A832-M5x10mm-Countersink:17
- Flush:72: CNC-005-XAxisMount1:1 ↔ 91263A832-M5x10mm-Countersink:19
- Mate:121: DSG16H-BallScrewFixtureBlock:2 ↔ CNC-006-XAxisMount2:1
- Mate:122: DSG16H-BallScrewFixtureBlock:2 ↔ CNC-006-XAxisMount2:1
- Mate:123: DSG16H-BallScrewFixtureBlock:2 ↔ CNC-006-XAxisMount2:1
- Mate:124: CNC-005-XAxisMount1:1 ↔ CNC-006-XAxisMount2:1
- Angle:7 (0 deg): CNC-005-XAxisMount1:1 ↔ CNC-006-XAxisMount2:1
- Mate:125: HGH20-LinearRailCarriage:7 ↔ CNC-006-XAxisMount2:1
- Mate:126: HGH20-LinearRailCarriage:7 ↔ CNC-006-XAxisMount2:1
- Mate:127: HGH20-LinearRailCarriage:7 ↔ CNC-006-XAxisMount2:1
- Mate:128: HGH20-LinearRailCarriage:6 ↔ CNC-006-XAxisMount2:1
- Mate:129: HGH20-LinearRailCarriage:6 ↔ CNC-006-XAxisMount2:1
- Mate:130: HGH20-LinearRailCarriage:6 ↔ CNC-006-XAxisMount2:1
- Mate:131: HGH20-LinearRailCarriage:5 ↔ CNC-006-XAxisMount2:1
- Mate:132: HGH20-LinearRailCarriage:5 ↔ CNC-006-XAxisMount2:1
- Mate:133: HGH20-LinearRailCarriage:5 ↔ CNC-006-XAxisMount2:1
- Mate:134: HGH20-LinearRailCarriage:8 ↔ CNC-006-XAxisMount2:1
- Mate:135: HGH20-LinearRailCarriage:8 ↔ CNC-006-XAxisMount2:1
- Mate:136: HGH20-LinearRailCarriage:8 ↔ CNC-006-XAxisMount2:1
- Mate:137: HGH20-LinearRailCarriage:8 ↔ HGR20R-LinearRail500mm:3
- Mate:138: HGH20-LinearRailCarriage:8 ↔ HGR20R-LinearRail500mm:3
- Mate:139: SFU1605-BallScrewNut:2 ↔ 91274A131_M5x20mm:11
- Mate:140: SFU1605-BallScrewNut:2 ↔ 91274A131_M5x20mm:11
- Mate:141: SFU1605-BallScrewNut:2 ↔ 91274A131_M5x20mm:14
- Mate:142: SFU1605-BallScrewNut:2 ↔ 91274A131_M5x20mm:16
- Mate:143: SFU1605-BallScrewNut:2 ↔ 91274A131_M5x20mm:15
- Mate:144: SFU1605-BallScrewNut:2 ↔ 91274A131_M5x20mm:13
- Mate:145: SFU1605-BallScrewNut:2 ↔ 91274A131_M5x20mm:12
- Flush:73: 91274A131_M5x20mm:14 ↔ 91274A131_M5x20mm:16
- Flush:74: 91274A131_M5x20mm:11 ↔ 91274A131_M5x20mm:14
- Flush:75: 91274A131_M5x20mm:11 ↔ 91274A131_M5x20mm:15
- Flush:76: 91274A131_M5x20mm:12 ↔ 91274A131_M5x20mm:16
- Flush:77: 91274A131_M5x20mm:12 ↔ 91274A131_M5x20mm:13
- Mate:146: CNC-006-XAxisMount2:1 ↔ 91263A832-M5x10mm-Countersink:22
- Mate:147: CNC-006-XAxisMount2:1 ↔ 91263A832-M5x10mm-Countersink:23
- Mate:148: CNC-006-XAxisMount2:1 ↔ 91263A832-M5x10mm-Countersink:24
- Mate:149: CNC-006-XAxisMount2:1 ↔ 91263A832-M5x10mm-Countersink:21
- Flush:78: CNC-006-XAxisMount2:1 ↔ 91263A832-M5x10mm-Countersink:21
- Flush:79: CNC-006-XAxisMount2:1 ↔ 91263A832-M5x10mm-Countersink:23
- Flush:80: 91263A832-M5x10mm-Countersink:22 ↔ 91263A832-M5x10mm-Countersink:23
- Flush:81: CNC-006-XAxisMount2:1 ↔ 91263A832-M5x10mm-Countersink:24
- Mate:150: CNC-006-XAxisMount2:1 ↔ 91263A832-M5x10mm-Countersink:25
- Mate:151: CNC-006-XAxisMount2:1 ↔ 91263A832-M5x10mm-Countersink:27
- Mate:152: CNC-006-XAxisMount2:1 ↔ 91263A832-M5x10mm-Countersink:28
- Mate:153: CNC-006-XAxisMount2:1 ↔ 91263A832-M5x10mm-Countersink:26
- Flush:82: CNC-006-XAxisMount2:1 ↔ 91263A832-M5x10mm-Countersink:27
- Flush:83: CNC-006-XAxisMount2:1 ↔ 91263A832-M5x10mm-Countersink:26
- Flush:84: CNC-006-XAxisMount2:1 ↔ 91263A832-M5x10mm-Countersink:28
- Flush:85: CNC-006-XAxisMount2:1 ↔ 91263A832-M5x10mm-Countersink:25
- Mate:154: CNC-006-XAxisMount2:1 ↔ 91263A832-M5x10mm-Countersink:31
- Mate:155: CNC-006-XAxisMount2:1 ↔ 91263A832-M5x10mm-Countersink:30
- Mate:156: CNC-006-XAxisMount2:1 ↔ 91263A832-M5x10mm-Countersink:29
- Mate:157: CNC-006-XAxisMount2:1 ↔ 91263A832-M5x10mm-Countersink:32
- Flush:86: CNC-006-XAxisMount2:1 ↔ 91263A832-M5x10mm-Countersink:32
- Flush:87: CNC-006-XAxisMount2:1 ↔ 91263A832-M5x10mm-Countersink:29
- Flush:88: 91263A832-M5x10mm-Countersink:29 ↔ 91263A832-M5x10mm-Countersink:31
- Flush:89: 91263A832-M5x10mm-Countersink:30 ↔ 91263A832-M5x10mm-Countersink:31
- Mate:158: CNC-006-XAxisMount2:1 ↔ 91263A832-M5x10mm-Countersink:35
- Mate:159: CNC-006-XAxisMount2:1 ↔ 91263A832-M5x10mm-Countersink:33
- Mate:160: CNC-006-XAxisMount2:1 ↔ 91263A832-M5x10mm-Countersink:34
- Mate:161: CNC-006-XAxisMount2:1 ↔ 91263A832-M5x10mm-Countersink:36
- Flush:90: CNC-006-XAxisMount2:1 ↔ 91263A832-M5x10mm-Countersink:36
- Flush:91: CNC-006-XAxisMount2:1 ↔ 91263A832-M5x10mm-Countersink:34
- Flush:92: CNC-006-XAxisMount2:1 ↔ 91263A832-M5x10mm-Countersink:35
- Flush:93: CNC-006-XAxisMount2:1 ↔ 91263A832-M5x10mm-Countersink:33
- Mate:162: CNC-006-XAxisMount2:1 ↔ 91263A832-M5x10mm-Countersink:38
- Mate:163: CNC-006-XAxisMount2:1 ↔ 91263A832-M5x10mm-Countersink:39
- Mate:164: CNC-006-XAxisMount2:1 ↔ 91263A832-M5x10mm-Countersink:37
- Mate:165: CNC-006-XAxisMount2:1 ↔ 91263A832-M5x10mm-Countersink:40
- Flush:94: CNC-006-XAxisMount2:1 ↔ 91263A832-M5x10mm-Countersink:40
- Flush:95: CNC-006-XAxisMount2:1 ↔ 91263A832-M5x10mm-Countersink:37
- Flush:96: CNC-006-XAxisMount2:1 ↔ 91263A832-M5x10mm-Countersink:38
- Flush:97: CNC-006-XAxisMount2:1 ↔ 91263A832-M5x10mm-Countersink:39
- Mate:166: CNC-005-XAxisMount1:1 ↔ CNC-006-XAxisMount2:1
- Mate:167: CNC-006-XAxisMount2:1 ↔ 92095A495-M8-18mm-ButtonHead:1
- Mate:168: CNC-006-XAxisMount2:1 ↔ 92095A495-M8-18mm-ButtonHead:2
- Mate:169: CNC-006-XAxisMount2:1 ↔ 92095A495-M8-18mm-ButtonHead:3
- Mate:170: CNC-006-XAxisMount2:1 ↔ 92095A495-M8-18mm-ButtonHead:3
- Flush:98: 92095A495-M8-18mm-ButtonHead:1 ↔ 92095A495-M8-18mm-ButtonHead:3
- Flush:99: 92095A495-M8-18mm-ButtonHead:1 ↔ 92095A495-M8-18mm-ButtonHead:2
- Mate:171: CNC-006-XAxisMount2:1 ↔ 92095A495-M8-18mm-ButtonHead:8
- Flush:100: 92095A495-M8-18mm-ButtonHead:3 ↔ 92095A495-M8-18mm-ButtonHead:8
- Mate:172: CNC-006-XAxisMount2:1 ↔ 92095A495-M8-18mm-ButtonHead:11
- Mate:173: CNC-006-XAxisMount2:1 ↔ 92095A495-M8-18mm-ButtonHead:12
- Flush:101: 92095A495-M8-18mm-ButtonHead:11 ↔ 92095A495-M8-18mm-ButtonHead:12
- Flush:102: 92095A495-M8-18mm-ButtonHead:1 ↔ 92095A495-M8-18mm-ButtonHead:11
- Mate:174: CNC-006-XAxisMount2:1 ↔ 92095A495-M8-18mm-ButtonHead:9
- Mate:175: CNC-006-XAxisMount2:1 ↔ 92095A495-M8-18mm-ButtonHead:10
- Flush:103: 92095A495-M8-18mm-ButtonHead:9 ↔ 92095A495-M8-18mm-ButtonHead:10